# Autodesk Inventor assembly: prototype
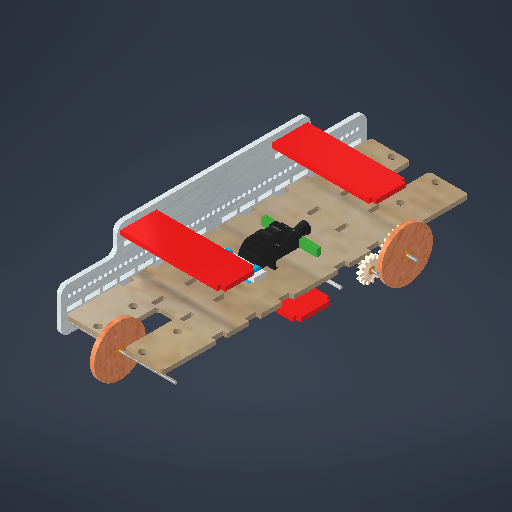
[picture p0: Inventor's stored thumbnail of the model, 512x512]
Saved by Autodesk Inventor 2025.3 (Build 293356030, 356C)
## iProperties
Created: 2025-09-04
Part Number: prototype
Document SubType Name: Assembly
Designer: 陳泓任
Author: 陳泓任
## Documents named in this file (14)
- C:\Users\Ou918\3D-model-temp\introduction to mechanical engineering(1)\version_3\prototype.iam
- C:\Users\Ou918\3D-model-temp\introduction to mechanical engineering(1)\發條組合\發條組合.iam
- C:\Users\Ou918\3D-model-temp\introduction to mechanical engineering(1)\side_frame.ipt
- C:\Users\Ou918\3D-model-temp\introduction to mechanical engineering(1)\version_2\plug.ipt
- C:\Users\Ou918\3D-model-temp\introduction to mechanical engineering(1)\beam.ipt
- C:\Users\Ou918\3D-model-temp\introduction to mechanical engineering(1)\80mm rod.ipt
- C:\Users\Ou918\3D-model-temp\introduction to mechanical engineering(1)\100mm rod.ipt
- C:\Users\Ou918\3D-model-temp\introduction to mechanical engineering(1)\big gear(with sleeve).iam
- C:\Users\Ou918\3D-model-temp\introduction to mechanical engineering(1)\small gear(with sleeve).iam
- C:\Users\Ou918\3D-model-temp\introduction to mechanical engineering(1)\35mm wheel(with sleeve).iam
- C:\Users\Ou918\3D-model-temp\introduction to mechanical engineering(1)\sleeve.ipt
- C:\Users\Ou918\3D-model-temp\introduction to mechanical engineering(1)\baffle.ipt
- C:\Users\Ou918\3D-model-temp\introduction to mechanical engineering(1)\version_2\main_frame.ipt
- C:\Users\Ou918\3D-model-temp\introduction to mechanical engineering(1)\support.ipt
## Components (24 placed, 13 different names)
1. main_frame:1 — x origin, side frame(right), 貼合:48, 貼合:49, 貼合:50, 貼合:51, 相切:1, 角度:1, wheel, rod(front), 貼合:83, 貼合:84, 貼合:85, 貼合:87, 貼合:91, 貼合:92
2. 發條組合:1 [sub-assembly] — hole, gear, 貼合:82, 貼合:90, 貼合:92, 貼合:93, 貼合:94
3. side_frame:1 — 齊平:1, 齊平:2, hole, 對稱:1, 貼合:24, 貼合:25, 貼合:29, 貼合:32, 貼合:37
4. side_frame:2 — 齊平:1, 齊平:2, side frame(right), 貼合:13, 貼合:14, 貼合:15, 貼合:16, 貼合:17, 貼合:18, 貼合:19, 貼合:20, 對稱:1, 插入:3
5. beam:1 — 齊平:3, 貼合:13, 貼合:14, 貼合:15
6. beam:2 — 齊平:3, 貼合:16, 貼合:17
7. beam:3 — 貼合:18, 貼合:19, 貼合:20
8. 80mm rod:1 — 貼合:29, 貼合:30
9. 100mm rod:1 — 貼合:21, 貼合:27, 貼合:32, 貼合:77
10. big gear(with sleeve):1 [sub-assembly] — gear, 齊平:4
11. big gear(with sleeve):2 [sub-assembly] — 貼合:21, 齊平:5, 貼合:78
12. small gear(with sleeve):1 [sub-assembly] — 貼合:30, 齊平:4, 齊平:5
13. 35mm wheel(with sleeve):2 [sub-assembly] — 插入:2
14. 35mm wheel(with sleeve):3 [sub-assembly] — 貼合:43, wheel
15. sleeve:1 — 插入:2, 插入:3
16. 80mm rod:2 — 貼合:37, 貼合:43, 相切:1, rod(front)
17. support:3 — 貼合:50, 貼合:51, 貼合:54, 貼合:75
18. support:4 — 貼合:48, 貼合:49, 貼合:53, 貼合:55, 貼合:56, 貼合:57, 貼合:58
19. baffle:1 — 貼合:53, 貼合:54, 貼合:55, 貼合:56, 貼合:94
20. baffle:2 — 貼合:57, 貼合:58, 貼合:75
21. baffle:3 — 貼合:86, 貼合:88, 貼合:89, 貼合:90, 貼合:91, 貼合:93
22. plug:3 — 貼合:83, 貼合:84, 貼合:85, 貼合:86
23. plug:4 — 貼合:87, 貼合:88, 貼合:89
24. 35mm wheel(with sleeve):4 [sub-assembly] — 貼合:77, 貼合:78
## Relationships (59: Mate 48, Flush 5, Insert 3, Symmetry 1, Tangent 1, Angle 1)
- 齊平:1 [Flush]: side_frame:1 ↔ side_frame:2
- 齊平:2 [Flush]: side_frame:1 ↔ side_frame:2
- hole [Mate]: 發條組合:1 ↔ side_frame:1
- x origin [Mate]: main_frame:1
- side frame(right) [Mate]: main_frame:1 ↔ side_frame:2
- 齊平:3 [Flush]: beam:1 ↔ beam:2
- 貼合:13 [Mate]: side_frame:2 ↔ beam:1
- 貼合:14 [Mate]: side_frame:2 ↔ beam:1
- 貼合:15 [Mate]: side_frame:2 ↔ beam:1
- 貼合:16 [Mate]: side_frame:2 ↔ beam:2
- 貼合:17 [Mate]: side_frame:2 ↔ beam:2
- 貼合:18 [Mate]: side_frame:2 ↔ beam:3
- 貼合:19 [Mate]: side_frame:2 ↔ beam:3
- 貼合:20 [Mate]: side_frame:2 ↔ beam:3
- 貼合:21 [Mate]: 100mm rod:1 ↔ big gear(with sleeve):2
- 對稱:1 [Symmetry]: side_frame:1 ↔ side_frame:2
- 貼合:24 [Mate]: side_frame:1
- 貼合:25 [Mate]: side_frame:1
- 貼合:27 [Mate] (50 mm): 100mm rod:1
- gear [Insert]: 發條組合:1 ↔ big gear(with sleeve):1
- 貼合:29 [Mate]: side_frame:1 ↔ 80mm rod:1
- 貼合:30 [Mate]: 80mm rod:1 ↔ small gear(with sleeve):1
- 齊平:4 [Flush]: big gear(with sleeve):1 ↔ small gear(with sleeve):1
- 齊平:5 [Flush]: big gear(with sleeve):2 ↔ small gear(with sleeve):1
- 貼合:32 [Mate]: side_frame:1 ↔ 100mm rod:1
- 插入:2 [Insert]: 35mm wheel(with sleeve):2 ↔ sleeve:1
- 插入:3 [Insert]: side_frame:2 ↔ sleeve:1
- 貼合:37 [Mate]: side_frame:1 ↔ 80mm rod:2
- 貼合:43 [Mate]: 35mm wheel(with sleeve):3 ↔ 80mm rod:2
- 貼合:48 [Mate]: main_frame:1 ↔ support:4
- 貼合:49 [Mate]: main_frame:1 ↔ support:4
- 貼合:50 [Mate]: main_frame:1 ↔ support:3
- 貼合:51 [Mate]: main_frame:1 ↔ support:3
- 貼合:53 [Mate]: support:4 ↔ baffle:1
- 貼合:54 [Mate]: support:3 ↔ baffle:1
- 貼合:55 [Mate]: support:4 ↔ baffle:1
- 貼合:56 [Mate]: support:4 ↔ baffle:1
- 貼合:57 [Mate]: support:4 ↔ baffle:2
- 貼合:58 [Mate]: support:4 ↔ baffle:2
- 相切:1 [Tangent]: main_frame:1 ↔ 80mm rod:2
- 角度:1 [Angle] (90 deg): main_frame:1
- 貼合:75 [Mate]: support:3 ↔ baffle:2
- 貼合:77 [Mate]: 100mm rod:1 ↔ 35mm wheel(with sleeve):4
- 貼合:78 [Mate]: big gear(with sleeve):2 ↔ 35mm wheel(with sleeve):4
- wheel [Mate] (5 mm): main_frame:1 ↔ 35mm wheel(with sleeve):3
- rod(front) [Mate] (40 mm): main_frame:1 ↔ 80mm rod:2
- 貼合:82 [Mate] (-6.75 mm): 發條組合:1
- 貼合:83 [Mate]: main_frame:1 ↔ plug:3
- 貼合:84 [Mate]: main_frame:1 ↔ plug:3
- 貼合:85 [Mate]: main_frame:1 ↔ plug:3
- 貼合:86 [Mate]: baffle:3 ↔ plug:3
- 貼合:87 [Mate]: main_frame:1 ↔ plug:4
- 貼合:88 [Mate]: baffle:3 ↔ plug:4
- 貼合:89 [Mate]: baffle:3 ↔ plug:4
- 貼合:90 [Mate]: 發條組合:1 ↔ baffle:3
- 貼合:91 [Mate]: main_frame:1 ↔ baffle:3
- 貼合:92 [Mate]: main_frame:1 ↔ 發條組合:1
- 貼合:93 [Mate]: 發條組合:1 ↔ baffle:3
- 貼合:94 [Mate]: 發條組合:1 ↔ baffle:1
